# Autodesk Inventor assembly: ManualClamp
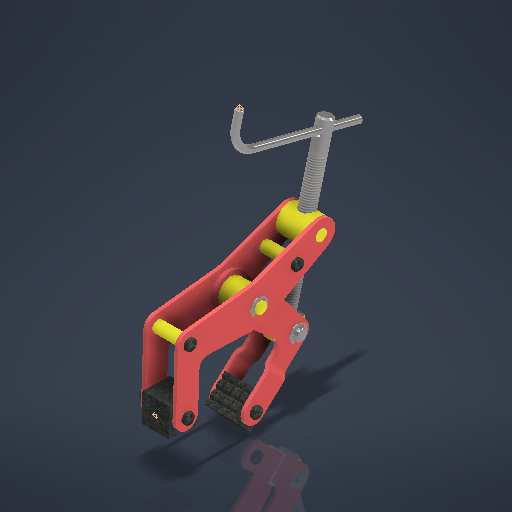
[picture p0: Inventor's stored thumbnail of the model, 512x512]
Saved by Autodesk Inventor 2025.4 (Build 294407000, 407)
## iProperties
Created: 2026-05-27
Part Number: ManualClamp
Document SubType Name: Assembly
Designer: VuQuan
Author: VuQuan
## Documents named in this file (15)
- D:\Edu\4CHaUI-Inventor\Assembly\b1\clamp\ManualClamp.iam
- D:\Edu\4CHaUI-Inventor\Assembly\b1\clamp\Base.ipt
- D:\Edu\4CHaUI-Inventor\Assembly\b1\clamp\BaseSpacer.ipt
- D:\Edu\4CHaUI-Inventor\Assembly\b1\clamp\BaseSupport.ipt
- D:\Edu\4CHaUI-Inventor\Assembly\b1\clamp\Elbow.ipt
- D:\Edu\4CHaUI-Inventor\Assembly\b1\clamp\Foot.ipt
- D:\Edu\4CHaUI-Inventor\Assembly\b1\clamp\FootPin.ipt
- D:\Edu\4CHaUI-Inventor\Assembly\b1\clamp\Hinge.ipt
- D:\Edu\4CHaUI-Inventor\Assembly\b1\clamp\Lever.ipt
- D:\Edu\4CHaUI-Inventor\Assembly\b1\clamp\Rod.ipt
- D:\Edu\4CHaUI-Inventor\Assembly\b1\clamp\Tee.ipt
- D:\Edu\4CHaUI-Inventor\Assembly\b1\clamp\Elbow_MIR.ipt
- C:\Users\VuQuan\OneDrive\Tài liệu\Inventor\Content Center Files\R2025\en-US\DIN 6799\DIN 6799 - 5 6.ipt
- C:\Users\VuQuan\OneDrive\Tài liệu\Inventor\Content Center Files\R2025\en-US\DIN 6799\DIN 6799 - 6 7.ipt
- C:\Users\VuQuan\OneDrive\Tài liệu\Inventor\Content Center Files\R2025\en-US\ISO 7045  H\ISO 7045 - M4 x 10_ - 4.8 - H - ISO.ipt
## Components (28 placed, 14 different names)
1. Base:1 — Insert:3, Insert:5, Mate:2, Insert:7, Insert:9, Insert:10, Mate:9, Mate:15, Mate:17, Mate:18
2. BaseSpacer:1 — Insert:5, Insert:6, Mate:4
3. BaseSupport:1 — Insert:9
4. Elbow:1 — Insert:1, Insert:3, Mate:6, Mate:16, Angle:2
5. Foot:1 — Mate:8, Mate:9, Angle:1
6. FootPin:1 — Insert:7, Mate:8
7. Hinge:1 — Insert:1, Insert:2, Insert:12, Insert:15
8. Lever:1 — Mate:14, Angle:6
9. Rod:1 — Mate:4, Mate:12, Insert:11, Mate:14, Angle:5, Angle:6
10. Tee:1 — Mate:6, Mate:7, Mate:12, Mate:13, Insert:13, Insert:14, Angle:5
11. Base:2 — Insert:4, Insert:6, Insert:16, Insert:18, Insert:19, Angle:1, Angle:4
12. Elbow_MIR:1 — Insert:2, Insert:4, Mate:7, Insert:8, Mate:11, Angle:4
13. FootPin:2 — Insert:8, Mate:10, Insert:17
14. BaseSupport:2 — Insert:10
15. Foot:2 — Mate:10, Mate:11, Angle:2
16. DIN 6799 5:1 — Insert:11, Mate:13
17. DIN 6799 6:1 — Insert:13
18. DIN 6799 6:2 — Insert:15
19. DIN 6799 6:3 — Insert:12
20. DIN 6799 6:4 — Insert:14
21. ISO 7045 H M4 x 10 - 4.8 - H:1 — Insert:17
22. ISO 7045 H M4 x 10 - 4.8 - H:2 — Mate:16
23. ISO 7045 H M4 x 10 - 4.8 - H:3 — Insert:18
24. ISO 7045 H M4 x 10 - 4.8 - H:4 — Insert:19
25. ISO 7045 H M4 x 10 - 4.8 - H:5 — Mate:18
26. ISO 7045 H M4 x 10 - 4.8 - H:6 — Mate:17
27. ISO 7045 H M4 x 10 - 4.8 - H:7 — Mate:15
28. ISO 7045 H M4 x 10 - 4.8 - H:8 — Insert:16
## Relationships (39: Insert 19, Mate 15, Angle 5)
- Insert:1: Elbow:1 ↔ Hinge:1
- Insert:2: Hinge:1 ↔ Elbow_MIR:1
- Insert:3: Base:1 ↔ Elbow:1
- Insert:4: Base:2 ↔ Elbow_MIR:1
- Insert:5: Base:1 ↔ BaseSpacer:1
- Insert:6: BaseSpacer:1 ↔ Base:2
- Mate:2: Base:1
- Mate:4: BaseSpacer:1 ↔ Rod:1
- Mate:6: Elbow:1 ↔ Tee:1
- Mate:7: Tee:1 ↔ Elbow_MIR:1
- Insert:7: Base:1 ↔ FootPin:1
- Insert:8: Elbow_MIR:1 ↔ FootPin:2
- Insert:9: Base:1 ↔ BaseSupport:1
- Insert:10: Base:1 ↔ BaseSupport:2
- Mate:8: Foot:1 ↔ FootPin:1
- Mate:9 (0.2 mm): Base:1 ↔ Foot:1
- Mate:10: FootPin:2 ↔ Foot:2
- Mate:11 (0.2 mm): Elbow_MIR:1 ↔ Foot:2
- Mate:12: Rod:1 ↔ Tee:1
- Insert:11: Rod:1 ↔ DIN 6799 5:1
- Mate:13: Tee:1 ↔ DIN 6799 5:1
- Insert:12: Hinge:1 ↔ DIN 6799 6:3
- Insert:13: Tee:1 ↔ DIN 6799 6:1
- Insert:14: Tee:1 ↔ DIN 6799 6:4
- Insert:15: Hinge:1 ↔ DIN 6799 6:2
- Mate:14: Lever:1 ↔ Rod:1
- Insert:16: Base:2 ↔ ISO 7045 H M4 x 10 - 4.8 - H:8
- Insert:17: FootPin:2 ↔ ISO 7045 H M4 x 10 - 4.8 - H:1
- Insert:18: Base:2 ↔ ISO 7045 H M4 x 10 - 4.8 - H:3
- Insert:19: Base:2 ↔ ISO 7045 H M4 x 10 - 4.8 - H:4
- Mate:15: Base:1 ↔ ISO 7045 H M4 x 10 - 4.8 - H:7
- Mate:16: Elbow:1 ↔ ISO 7045 H M4 x 10 - 4.8 - H:2
- Mate:17: Base:1 ↔ ISO 7045 H M4 x 10 - 4.8 - H:6
- Mate:18: Base:1 ↔ ISO 7045 H M4 x 10 - 4.8 - H:5
- Angle:1 (0 deg): Foot:1 ↔ Base:2
- Angle:2 (0 deg): Elbow:1 ↔ Foot:2
- Angle:4 (-40 deg): Base:2 ↔ Elbow_MIR:1
- Angle:5 (0 deg): Rod:1 ↔ Tee:1
- Angle:6 (0 deg): Lever:1 ↔ Rod:1
